# Autodesk Inventor assembly: driving motors
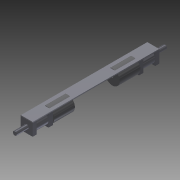
[picture p0: Inventor's stored thumbnail of the model, 180x180]
Saved by Autodesk Inventor 2011 (Build 150239000, 239)
## iProperties
Created: 2013-01-19
Part Number: driving motors
Document SubType Name: Assembly
Designer: Christopher
Author: Christopher
## Documents named in this file (4)
- F:\Users\Christopher\Documents\GitHub\2013CAD\2013 robot\forklift\Pneumatics and frame grabbers\driving motors.iam
- F:\Users\Christopher\Documents\GitHub\2013CAD\2013 robot\forklift\Misc parts\hack_p60.ipt
- F:\Users\Christopher\Documents\GitHub\2013CAD\2013 robot\forklift\Misc parts\hack_775_motor.ipt
- F:\Users\Christopher\Documents\GitHub\2013CAD\2013 robot\forklift\Misc parts\steel_p60_mounting _plate.ipt
## Components (5 placed, 3 different names)
1. hack_p60:1 — Insert:1, Mate:1, Flush:1, Flush:2
2. hack_775_motor:1 — Insert:1
3. steel_p60_mounting _plate:1 — Mate:1, Flush:1, Flush:2, Mate:2, Flush:3, Flush:4
4. hack_775_motor:2 — Insert:2
5. hack_p60:2 — Insert:2, Mate:2, Flush:3, Flush:4
## Relationships (8: Flush 4, Insert 2, Mate 2)
- Insert:1: hack_p60:1 ↔ hack_775_motor:1
- Mate:1: hack_p60:1 ↔ steel_p60_mounting _plate:1
- Flush:1: hack_p60:1 ↔ steel_p60_mounting _plate:1
- Flush:2: hack_p60:1 ↔ steel_p60_mounting _plate:1
- Insert:2: hack_775_motor:2 ↔ hack_p60:2
- Mate:2: steel_p60_mounting _plate:1 ↔ hack_p60:2
- Flush:3: steel_p60_mounting _plate:1 ↔ hack_p60:2
- Flush:4: steel_p60_mounting _plate:1 ↔ hack_p60:2
